# Autodesk Inventor assembly: Boxbeam
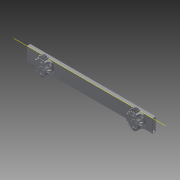
[picture p0: Inventor's stored thumbnail of the model, 180x180]
Saved by Autodesk Inventor 2015 (Build 190159000, 159)
## iProperties
Created: 2015-01-30
Part Number: Boxbeam
Document SubType Name: Assembly
Designer: chapale16
Author: chapale16
## Documents named in this file (3)
- \\lhssvr02\Homedirs\Robotics Club\CAD Model 2015\Box Beam Drive Base\Newest\Boxbeam.iam
- \\lhssvr02\Homedirs\Robotics Club\CAD Model 2015\Box Beam Drive Base\Newest\4x1 boxbeam lengths.ipt
- \\lhssvr02\Homedirs\Robotics Club\CAD Model 2015\Box Beam Drive Base\Newest\Toughbox-mini (1).iam
## Components (3 placed, 2 different names)
1. 4x1 boxbeam lengths:1 — Mate:1, Mate:6
2. Toughbox-mini (1):1 [sub-assembly] — Mate:1
3. Toughbox-mini (1):2 [sub-assembly] — Mate:6
## Relationships (2: Mate 2)
- Mate:1: 4x1 boxbeam lengths:1 ↔ Toughbox-mini (1):1
- Mate:6: 4x1 boxbeam lengths:1 ↔ Toughbox-mini (1):2
